# Autodesk Inventor assembly: Baugruppe9
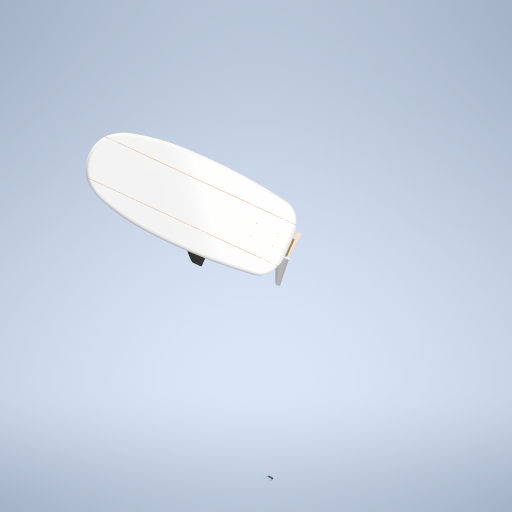
[picture p0: Inventor's stored thumbnail of the model, 512x512]
Saved by Autodesk Inventor 2024 (Build 280153000, 153)
## iProperties
Created: 2025-04-05
Part Number: Baugruppe9
Document SubType Name: Assembly
Designer: fynnb
Author: fynnb
## Documents named in this file (14)
- C:\Users\fynnb\Documents\Bachelorarbeit\Github Datein\CAD_Konstruktionen\Baugruppe9.iam
- C:\Users\fynnb\Documents\Bachelorarbeit\CAD\Efoil 2021-v1\CAD_Vorlage\Fästplatta v2.ipt
- C:\Users\fynnb\Documents\Bachelorarbeit\CAD\Efoil 2021-v1\CAD_Vorlage\Stainless Steel-Hinge GN 337-NI-40-40-A-1-GS(0)\Hinge GN 337-NI-40-40-A-1-GS-1.ipt
- C:\Users\fynnb\Documents\Bachelorarbeit\CAD\Efoil 2021-v1\CAD_Vorlage\Stainless Steel-Hinge GN 337-NI-40-40-A-1-GS(0)\Hinge GN 337-NI-40-40-A-1-GS-2.ipt
- C:\Users\fynnb\Documents\Bachelorarbeit\CAD\Efoil 2021-v1\CAD_Vorlage\Bauteil unten.ipt
- C:\Users\fynnb\Documents\Bachelorarbeit\CAD\Efoil 2021-v1\CAD_Vorlage\Mast efoil.ipt
- C:\Users\fynnb\Documents\Bachelorarbeit\CAD\Efoil 2021-v1\CAD_Vorlage\FUSELAGE v2.ipt
- C:\Users\fynnb\Documents\Bachelorarbeit\CAD\Efoil 2021-v1\CAD_Vorlage\Part35.ipt
- C:\Users\fynnb\Documents\Bachelorarbeit\CAD\Efoil 2021-v1\CAD_Vorlage\Frontvinge gong.ipt
- C:\Users\fynnb\Documents\Bachelorarbeit\CAD\Efoil 2021-v1\CAD_Vorlage\Bräda.iam
- C:\Users\fynnb\Documents\Bachelorarbeit\CAD\Efoil 2021-v1\CAD_Vorlage\57.4-45-74-B-SW.ipt
- C:\Users\fynnb\Documents\Bachelorarbeit\CAD\Efoil 2021-v1\CAD_Vorlage\Spiral retaining cable GN 111.4-50-14_TOP.iam
- C:\Users\fynnb\Documents\Bachelorarbeit\CAD\Efoil 2021-v1\CAD_Vorlage\Spiral retaining cable GN 111.4-50-14-2.ipt
- C:\Users\fynnb\Documents\Bachelorarbeit\CAD\Efoil 2021-v1\CAD_Vorlage\Gegenstück_Magnet.ipt
## Components (16 placed, 13 different names)
1. Fästplatta v2:1 — Starr:4, Passend:16, Passend:17, Passend:18, Passend:19, Passend:22, Passend:23, Passend:24, Winkel:1
2. Hinge GN 337-NI-40-40-A-1-GS-1:1 — Passend:16, Passend:17
3. Hinge GN 337-NI-40-40-A-1-GS-1:2 — Passend:18, Passend:19, Passend:20, Passend:21
4. Hinge GN 337-NI-40-40-A-1-GS-2:1 — Passend:15, Starr:5, Kugelförmig:2
5. Hinge GN 337-NI-40-40-A-1-GS-2:2 — Passend:13, Passend:14, Passend:20, Passend:21
6. Bauteil unten:1 — Passend:10, Passend:11, Passend:12, Passend:13, Passend:14, Passend:15, Starr:5, Winkel:1, Drehbar:2, Passend:25
7. Mast efoil:1 — Starr:3, Starr:4
8. FUSELAGE v2:1 — Starr:1, Starr:2, Starr:3
9. Part35:1 — Starr:2
10. Frontvinge gong:1 — Starr:1
11. Bräda:1 [sub-assembly] — Passend:10, Passend:11, Passend:12
12. 57.4-45-74-B-SW:1 — Passend:22, Passend:23, Passend:24
13. Spiral retaining cable GN 111.4-50-14_TOP:1 [sub-assembly]
14. Spiral retaining cable GN 111.4-50-14-2:1 — Drehbar:1
15. Spiral retaining cable GN 111.4-50-14-2:2 — Kugelförmig:2, Drehbar:1
16. Gegenstück_Magnet:1 — Drehbar:2, Passend:25
## Relationships (25: Mate 16, WeldJoint 5, RevoluteJoint 2, Angle 1, BallJoint 1)
- Starr:1 [WeldJoint]: FUSELAGE v2:1 ↔ Frontvinge gong:1
- Passend:10 [Mate]: Bauteil unten:1 ↔ Bräda:1
- Passend:11 [Mate]: Bauteil unten:1 ↔ Bräda:1
- Passend:12 [Mate]: Bauteil unten:1 ↔ Bräda:1
- Starr:2 [WeldJoint]: FUSELAGE v2:1 ↔ Part35:1
- Starr:3 [WeldJoint]: Mast efoil:1 ↔ FUSELAGE v2:1
- Starr:4 [WeldJoint]: Fästplatta v2:1 ↔ Mast efoil:1
- Passend:13 [Mate]: Hinge GN 337-NI-40-40-A-1-GS-2:2 ↔ Bauteil unten:1
- Passend:14 [Mate]: Hinge GN 337-NI-40-40-A-1-GS-2:2 ↔ Bauteil unten:1
- Passend:15 [Mate]: Hinge GN 337-NI-40-40-A-1-GS-2:1 ↔ Bauteil unten:1
- Starr:5 [WeldJoint]: Hinge GN 337-NI-40-40-A-1-GS-2:1 ↔ Bauteil unten:1
- Passend:16 [Mate]: Fästplatta v2:1 ↔ Hinge GN 337-NI-40-40-A-1-GS-1:1
- Passend:17 [Mate]: Fästplatta v2:1 ↔ Hinge GN 337-NI-40-40-A-1-GS-1:1
- Passend:18 [Mate]: Fästplatta v2:1 ↔ Hinge GN 337-NI-40-40-A-1-GS-1:2
- Passend:19 [Mate]: Fästplatta v2:1 ↔ Hinge GN 337-NI-40-40-A-1-GS-1:2
- Passend:20 [Mate]: Hinge GN 337-NI-40-40-A-1-GS-1:2 ↔ Hinge GN 337-NI-40-40-A-1-GS-2:2
- Passend:21 [Mate]: Hinge GN 337-NI-40-40-A-1-GS-1:2 ↔ Hinge GN 337-NI-40-40-A-1-GS-2:2
- Passend:22 [Mate]: Fästplatta v2:1 ↔ 57.4-45-74-B-SW:1
- Passend:23 [Mate]: Fästplatta v2:1 ↔ 57.4-45-74-B-SW:1
- Passend:24 [Mate]: Fästplatta v2:1 ↔ 57.4-45-74-B-SW:1
- Winkel:1 [Angle] (180 deg): Fästplatta v2:1 ↔ Bauteil unten:1
- Kugelförmig:2 [BallJoint]: Hinge GN 337-NI-40-40-A-1-GS-2:1 ↔ Spiral retaining cable GN 111.4-50-14-2:2
- Drehbar:1 [RevoluteJoint]: Spiral retaining cable GN 111.4-50-14-2:1 ↔ Spiral retaining cable GN 111.4-50-14-2:2
- Drehbar:2 [RevoluteJoint]: Bauteil unten:1 ↔ Gegenstück_Magnet:1
- Passend:25 [Mate]: Bauteil unten:1 ↔ Gegenstück_Magnet:1
## Named parameters: sa_0 = 30000
note: some values were not read from the file. Shown as the stored number, unit unknown: "sa_0".
